# Autodesk Inventor assembly: LiPol_module
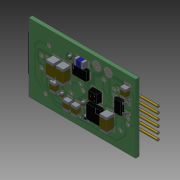
[picture p0: Inventor's stored thumbnail of the model, 180x180]
Saved by Autodesk Inventor 2013 (Build 170138000, 138)
## iProperties
Created: 2015-07-08
Part Number: LiPol_module
Document SubType Name: Assembly
Designer: terg
Author: terg
## Documents named in this file (16)
- C:\Users\terg\Projects\ModularElectronics\3D_models\LiPol_module\LiPol_module.iam
- C:\Users\terg\Projects\ModularElectronics\3D_models\LiPol_module\LiPol_module_PCB.ipt
- C:\Users\terg\Projects\ModularElectronics\3D_models\LiPol_module\LTC4411.ipt
- C:\Users\terg\Projects\ModularElectronics\3D_models\Components\0402_cap.ipt
- C:\Users\terg\Projects\ModularElectronics\3D_models\Components\0402_res.ipt
- C:\Users\terg\Projects\ModularElectronics\3D_models\Components\0603_led.ipt
- C:\Users\terg\Projects\ModularElectronics\3D_models\Components\0805_cap.ipt
- C:\Users\terg\Projects\ModularElectronics\3D_models\Components\EFM32ZG110.ipt
- C:\Users\terg\Projects\ModularElectronics\3D_models\Components\FemalConnector.ipt
- C:\Users\terg\Projects\ModularElectronics\3D_models\Components\MaleConnector.ipt
- C:\Users\terg\Projects\ModularElectronics\3D_models\Components\0805_res.ipt
- C:\Users\terg\Projects\ModularElectronics\3D_models\LiPol_module\ADP2504.ipt
- C:\Users\terg\Projects\ModularElectronics\3D_models\LiPol_module\ADP5063.ipt
- C:\Users\terg\Projects\ModularElectronics\3D_models\LiPol_module\LTC2942.ipt
- C:\Users\terg\Projects\ModularElectronics\3D_models\Components\1206_cap.ipt
- C:\Users\terg\Projects\ModularElectronics\3D_models\LiPol_module\EPL2010-332ML.ipt
## Components (34 placed, 15 different names)
1. LiPol_module_PCB:1 — Zestawiający:1, Równoległy:1, Równoległy:2, Zestawiający:2, Zestawiający:3, Zestawiający:4, Zestawiający:5, Zestawiający:6, Zestawiający:7, Zestawiający:8, Zestawiający:9, Zestawiający:10, Zestawiający:11, Równoległy:3, Równoległy:4, Równoległy:5, Równoległy:6, Równoległy:7, Równoległy:8, Równoległy:9, Równoległy:10, Równoległy:11, Równoległy:12, Równoległy:13, Równoległy:14, Zestawiający:12, Zestawiający:13, Zestawiający:14, Zestawiający:15, Równoległy:15, Równoległy:16, Równoległy:17, Równoległy:18, Równoległy:19, Równoległy:20, Równoległy:21, Równoległy:22, Zestawiający:16, Równoległy:23, Równoległy:24, Zestawiający:17, Zestawiający:20, Równoległy:25, Równoległy:26, Równoległy:27, Równoległy:28, Zestawiający:21, Równoległy:29, Równoległy:30, Zestawiający:22, Zestawiający:23, Równoległy:31, Równoległy:32, Równoległy:33, Równoległy:34, Zestawiający:24, Zestawiający:25, Zestawiający:26, Równoległy:35, Równoległy:36, Równoległy:37, Równoległy:38, Równoległy:39, Równoległy:40, Zestawiający:27, Równoległy:41, Równoległy:42, Równoległy:43, Równoległy:44, Równoległy:45, Równoległy:46, Równoległy:47, Równoległy:48, Równoległy:49, Równoległy:50, Zestawiający:28, Równoległy:51, Równoległy:52, Zestawiający:29, Równoległy:53, Równoległy:54, Zestawiający:30, Równoległy:55, Równoległy:56, Zestawiający:31, Równoległy:57, Równoległy:58, Zestawiający:32, Zestawiający:33, Zestawiający:34, Równoległy:59, Równoległy:60, Równoległy:61, Równoległy:62, Równoległy:63, Równoległy:64, Zestawiający:35, Zestawiający:36, Zestawiający:37
2. LTC4411:1 — Zestawiający:1, Równoległy:1, Równoległy:2
3. 0402_cap:1 — Zestawiający:4, Równoległy:43, Równoległy:44
4. 0402_cap:2 — Zestawiający:3, Równoległy:45, Równoległy:46
5. 0402_cap:3 — Zestawiający:2, Równoległy:49, Równoległy:50
6. 0402_res:1 — Zestawiający:5, Równoległy:47, Równoległy:48
7. 0402_cap:4 — Zestawiający:9, Równoległy:5, Równoległy:11
8. 0402_cap:5 — Zestawiający:8, Równoległy:4, Równoległy:14
9. 0402_cap:6 — Zestawiający:6, Równoległy:6, Równoległy:12
10. 0402_cap:7 — Zestawiający:7, Równoległy:7, Równoległy:9
11. 0402_cap:8 — Zestawiający:10, Równoległy:8, Równoległy:10
12. 0402_cap:9 — Zestawiający:11, Równoległy:3, Równoległy:13
13. 0402_res:2 — Zestawiający:12, Równoległy:15, Równoległy:20
14. 0402_res:3 — Zestawiający:13, Równoległy:16, Równoległy:19
15. 0402_res:4 — Zestawiający:14, Równoległy:17, Równoległy:18
16. 0402_res:5 — Zestawiający:15, Równoległy:21, Równoległy:22
17. 0603_led:1 — Zestawiający:16, Równoległy:23, Równoległy:24
18. 0805_cap:1 — Zestawiający:17, Równoległy:25, Równoległy:26
19. 0805_cap:2 — Zestawiający:20, Równoległy:27, Równoległy:28
20. EFM32ZG110:1 — Zestawiający:21, Równoległy:29, Równoległy:30
21. FemalConnector:1 — Zestawiający:23, Równoległy:31, Równoległy:32
22. MaleConnector:1 — Zestawiający:22, Równoległy:33, Równoległy:34
23. 0805_cap:3 — Zestawiający:24, Równoległy:35, Równoległy:39
24. 0805_cap:4 — Zestawiający:25, Równoległy:37, Równoległy:40
25. 0805_cap:5 — Zestawiający:26, Równoległy:36, Równoległy:38
26. 0805_cap:6 — Zestawiający:27, Równoległy:41, Równoległy:42
27. 0805_res:1 — Zestawiający:28, Równoległy:51, Równoległy:52
28. ADP2504:1 — Zestawiający:29, Równoległy:53, Równoległy:54
29. ADP5063:1 — Zestawiający:30, Równoległy:55, Równoległy:56
30. LTC2942:1 — Zestawiający:31, Równoległy:57, Równoległy:58
31. 1206_cap:1 — Zestawiający:34, Równoległy:62, Równoległy:63
32. 1206_cap:2 — Zestawiający:33, Równoległy:59, Równoległy:60
33. 1206_cap:3 — Zestawiający:32, Równoległy:61, Równoległy:64
34. EPL2010-332ML:1 — Zestawiający:35, Zestawiający:36, Zestawiający:37
## Relationships (99: Flush 64, Mate 35)
- Zestawiający:1 [Mate]: LiPol_module_PCB:1 ↔ LTC4411:1
- Równoległy:1 [Flush] (7.524 mm): LiPol_module_PCB:1 ↔ LTC4411:1
- Równoległy:2 [Flush] (1.578 mm): LiPol_module_PCB:1 ↔ LTC4411:1
- Zestawiający:2 [Mate]: LiPol_module_PCB:1 ↔ 0402_cap:3
- Zestawiający:3 [Mate]: LiPol_module_PCB:1 ↔ 0402_cap:2
- Zestawiający:4 [Mate]: LiPol_module_PCB:1 ↔ 0402_cap:1
- Zestawiający:5 [Mate]: LiPol_module_PCB:1 ↔ 0402_res:1
- Zestawiający:6 [Mate]: LiPol_module_PCB:1 ↔ 0402_cap:6
- Zestawiający:7 [Mate]: LiPol_module_PCB:1 ↔ 0402_cap:7
- Zestawiający:8 [Mate]: LiPol_module_PCB:1 ↔ 0402_cap:5
- Zestawiający:9 [Mate]: LiPol_module_PCB:1 ↔ 0402_cap:4
- Zestawiający:10 [Mate]: LiPol_module_PCB:1 ↔ 0402_cap:8
- Zestawiający:11 [Mate]: LiPol_module_PCB:1 ↔ 0402_cap:9
- Równoległy:3 [Flush] (2.556 mm): LiPol_module_PCB:1 ↔ 0402_cap:9
- Równoległy:4 [Flush] (4.993 mm): LiPol_module_PCB:1 ↔ 0402_cap:5
- Równoległy:5 [Flush] (8.143 mm): LiPol_module_PCB:1 ↔ 0402_cap:4
- Równoległy:6 [Flush] (11.422 mm): LiPol_module_PCB:1 ↔ 0402_cap:6
- Równoległy:7 [Flush] (8.933 mm): LiPol_module_PCB:1 ↔ 0402_cap:7
- Równoległy:8 [Flush] (10.636 mm): LiPol_module_PCB:1 ↔ 0402_cap:8
- Równoległy:9 [Flush] (3.792 mm): LiPol_module_PCB:1 ↔ 0402_cap:7
- Równoległy:10 [Flush] (3.668 mm): LiPol_module_PCB:1 ↔ 0402_cap:8
- Równoległy:11 [Flush] (11.271 mm): LiPol_module_PCB:1 ↔ 0402_cap:4
- Równoległy:12 [Flush] (10.895 mm): LiPol_module_PCB:1 ↔ 0402_cap:6
- Równoległy:13 [Flush] (9.603 mm): LiPol_module_PCB:1 ↔ 0402_cap:9
- Równoległy:14 [Flush] (11.773 mm): LiPol_module_PCB:1 ↔ 0402_cap:5
- Zestawiający:12 [Mate]: LiPol_module_PCB:1 ↔ 0402_res:2
- Zestawiający:13 [Mate]: LiPol_module_PCB:1 ↔ 0402_res:3
- Zestawiający:14 [Mate]: LiPol_module_PCB:1 ↔ 0402_res:4
- Zestawiający:15 [Mate]: LiPol_module_PCB:1 ↔ 0402_res:5
- Równoległy:15 [Flush] (3.172 mm): LiPol_module_PCB:1 ↔ 0402_res:2
- Równoległy:16 [Flush] (3.655 mm): LiPol_module_PCB:1 ↔ 0402_res:3
- Równoległy:17 [Flush] (3.639 mm): LiPol_module_PCB:1 ↔ 0402_res:4
- Równoległy:18 [Flush] (11.542 mm): LiPol_module_PCB:1 ↔ 0402_res:4
- Równoległy:19 [Flush] (12.434 mm): LiPol_module_PCB:1 ↔ 0402_res:3
- Równoległy:20 [Flush] (14.552 mm): LiPol_module_PCB:1 ↔ 0402_res:2
- Równoległy:21 [Flush] (10.801 mm): LiPol_module_PCB:1 ↔ 0402_res:5
- Równoległy:22 [Flush] (13.96 mm): LiPol_module_PCB:1 ↔ 0402_res:5
- Zestawiający:16 [Mate]: LiPol_module_PCB:1 ↔ 0603_led:1
- Równoległy:23 [Flush] (5.938 mm): LiPol_module_PCB:1 ↔ 0603_led:1
- Równoległy:24 [Flush] (3.547 mm): LiPol_module_PCB:1 ↔ 0603_led:1
- Zestawiający:17 [Mate]: LiPol_module_PCB:1 ↔ 0805_cap:1
- Zestawiający:20 [Mate]: LiPol_module_PCB:1 ↔ 0805_cap:2
- Równoległy:25 [Flush] (5.155 mm): LiPol_module_PCB:1 ↔ 0805_cap:1
- Równoległy:26 [Flush] (3.032 mm): LiPol_module_PCB:1 ↔ 0805_cap:1
- Równoległy:27 [Flush] (12.454 mm): LiPol_module_PCB:1 ↔ 0805_cap:2
- Równoległy:28 [Flush] (1.348 mm): LiPol_module_PCB:1 ↔ 0805_cap:2
- Zestawiający:21 [Mate]: LiPol_module_PCB:1 ↔ EFM32ZG110:1
- Równoległy:29 [Flush] (5.111 mm): LiPol_module_PCB:1 ↔ EFM32ZG110:1
- Równoległy:30 [Flush] (4.996 mm): LiPol_module_PCB:1 ↔ EFM32ZG110:1
- Zestawiający:22 [Mate]: LiPol_module_PCB:1 ↔ MaleConnector:1
- Zestawiający:23 [Mate]: LiPol_module_PCB:1 ↔ FemalConnector:1
- Równoległy:31 [Flush] (3.529 mm): LiPol_module_PCB:1 ↔ FemalConnector:1
- Równoległy:32 [Flush] (-0.948 mm): LiPol_module_PCB:1 ↔ FemalConnector:1
- Równoległy:33 [Flush] (4.072 mm): LiPol_module_PCB:1 ↔ MaleConnector:1
- Równoległy:34 [Flush] (-3.406 mm): LiPol_module_PCB:1 ↔ MaleConnector:1
- Zestawiający:24 [Mate]: LiPol_module_PCB:1 ↔ 0805_cap:3
- Zestawiający:25 [Mate]: LiPol_module_PCB:1 ↔ 0805_cap:4
- Zestawiający:26 [Mate]: LiPol_module_PCB:1 ↔ 0805_cap:5
- Równoległy:35 [Flush] (2.176 mm): LiPol_module_PCB:1 ↔ 0805_cap:3
- Równoległy:36 [Flush] (2.192 mm): LiPol_module_PCB:1 ↔ 0805_cap:5
- Równoległy:37 [Flush] (4.232 mm): LiPol_module_PCB:1 ↔ 0805_cap:4
- Równoległy:38 [Flush] (8.397 mm): LiPol_module_PCB:1 ↔ 0805_cap:5
- Równoległy:39 [Flush] (10.162 mm): LiPol_module_PCB:1 ↔ 0805_cap:3
- Równoległy:40 [Flush] (5.449 mm): LiPol_module_PCB:1 ↔ 0805_cap:4
- Zestawiający:27 [Mate]: LiPol_module_PCB:1 ↔ 0805_cap:6
- Równoległy:41 [Flush] (1.212 mm): LiPol_module_PCB:1 ↔ 0805_cap:6
- Równoległy:42 [Flush] (2.12 mm): LiPol_module_PCB:1 ↔ 0805_cap:6
- Równoległy:43 [Flush] (2.391 mm): LiPol_module_PCB:1 ↔ 0402_cap:1
- Równoległy:44 [Flush] (9.002 mm): LiPol_module_PCB:1 ↔ 0402_cap:1
- Równoległy:45 [Flush] (4.32 mm): LiPol_module_PCB:1 ↔ 0402_cap:2
- Równoległy:46 [Flush] (11.007 mm): LiPol_module_PCB:1 ↔ 0402_cap:2
- Równoległy:47 [Flush] (2.049 mm): LiPol_module_PCB:1 ↔ 0402_res:1
- Równoległy:48 [Flush] (10.344 mm): LiPol_module_PCB:1 ↔ 0402_res:1
- Równoległy:49 [Flush] (3.658 mm): LiPol_module_PCB:1 ↔ 0402_cap:3
- Równoległy:50 [Flush] (7.268 mm): LiPol_module_PCB:1 ↔ 0402_cap:3
- Zestawiający:28 [Mate]: LiPol_module_PCB:1 ↔ 0805_res:1
- Równoległy:51 [Flush] (10.559 mm): LiPol_module_PCB:1 ↔ 0805_res:1
- Równoległy:52 [Flush] (1.714 mm): LiPol_module_PCB:1 ↔ 0805_res:1
- Zestawiający:29 [Mate]: LiPol_module_PCB:1 ↔ ADP2504:1
- Równoległy:53 [Flush] (3.007 mm): LiPol_module_PCB:1 ↔ ADP2504:1
- Równoległy:54 [Flush] (6.938 mm): LiPol_module_PCB:1 ↔ ADP2504:1
- Zestawiający:30 [Mate]: LiPol_module_PCB:1 ↔ ADP5063:1
- Równoległy:55 [Flush] (5.254 mm): LiPol_module_PCB:1 ↔ ADP5063:1
- Równoległy:56 [Flush] (5.614 mm): LiPol_module_PCB:1 ↔ ADP5063:1
- Zestawiający:31 [Mate]: LiPol_module_PCB:1 ↔ LTC2942:1
- Równoległy:57 [Flush] (3.204 mm): LiPol_module_PCB:1 ↔ LTC2942:1
- Równoległy:58 [Flush] (10.132 mm): LiPol_module_PCB:1 ↔ LTC2942:1
- Zestawiający:32 [Mate]: LiPol_module_PCB:1 ↔ 1206_cap:3
- Zestawiający:33 [Mate]: LiPol_module_PCB:1 ↔ 1206_cap:2
- Zestawiający:34 [Mate]: LiPol_module_PCB:1 ↔ 1206_cap:1
- Równoległy:59 [Flush] (2.942 mm): LiPol_module_PCB:1 ↔ 1206_cap:2
- Równoległy:60 [Flush] (4.707 mm): LiPol_module_PCB:1 ↔ 1206_cap:2
- Równoległy:61 [Flush] (7.321 mm): LiPol_module_PCB:1 ↔ 1206_cap:3
- Równoległy:62 [Flush] (7.322 mm): LiPol_module_PCB:1 ↔ 1206_cap:1
- Równoległy:63 [Flush] (5.375 mm): LiPol_module_PCB:1 ↔ 1206_cap:1
- Równoległy:64 [Flush] (7.546 mm): LiPol_module_PCB:1 ↔ 1206_cap:3
- Zestawiający:35 [Mate]: LiPol_module_PCB:1 ↔ EPL2010-332ML:1
- Zestawiający:36 [Mate] (7.427 mm): LiPol_module_PCB:1 ↔ EPL2010-332ML:1
- Zestawiający:37 [Mate] (6.28 mm): LiPol_module_PCB:1 ↔ EPL2010-332ML:1
